# Autodesk Inventor assembly: Imaging System
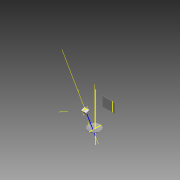
[picture p0: Inventor's stored thumbnail of the model, 180x180]
Saved by Autodesk Inventor 2012 (Build 160160000, 160)
## iProperties
Created: 2012-11-23
Part Number: Imaging System
Document SubType Name: Assembly
Designer: r0oland
Author: r0oland
## Documents named in this file (4)
- X:\Cloud Drives\Dropbox\Europhotonics\Personal Project\Inventor\Imaging System.iam
- X:\Cloud Drives\Dropbox\Europhotonics\Personal Project\Inventor\Mirror.ipt
- X:\Cloud Drives\Dropbox\Europhotonics\Personal Project\Inventor\camera.ipt
- X:\Cloud Drives\Dropbox\Europhotonics\Personal Project\Inventor\screen.ipt
## Components (3 placed, 3 different names)
1. Mirror:1 — Mate:1
2. camera:1 — Mate:2, Mate:3, Mate:4, Mate:5, Mate:6, Angle:1, Flush:1, Angle:3
3. screen:1 — Flush:1
## Relationships (14: Mate 10, Angle 3, Flush 1)
- Mate:1: Mirror:1
- Mate:2: camera:1
- Mate:3: camera:1
- Mate:4: camera:1
- Mate:5: camera:1
- Mate:6: camera:1
- Mate:7
- Mate:8
- Mate:9
- Angle:1 (0 deg): camera:1
- Angle:2 (20 deg)
- Flush:1: camera:1 ↔ screen:1
- Mate:10
- Angle:3 (0 deg): camera:1
